# Autodesk Inventor assembly: BedAssembly
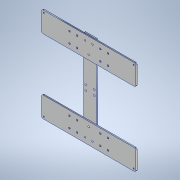
[picture p0: Inventor's stored thumbnail of the model, 180x180]
Saved by Autodesk Inventor 2020.2 (Build 242310000, 310)
## iProperties
Created: 2020-08-19
Part Number: BedAssembly
Document SubType Name: Assembly
Designer: JK
Author: JK
## Documents named in this file (3)
- C:\Users\JK\Documents\Inventor\Anet Upgrade\BedAssembly.iam
- C:\Users\JK\Documents\Inventor\Anet Upgrade\BedCarriageA.ipt
- C:\Users\JK\Documents\Inventor\Anet Upgrade\BedCarriageB.ipt
## Components (2 placed, 2 different names)
1. BedCarriageA:1 — Mate:1, Mate:2, Flush:1
2. BedCarriageB:1 — Mate:1, Mate:2, Flush:1
## Relationships (3: Mate 2, Flush 1)
- Mate:1: BedCarriageA:1 ↔ BedCarriageB:1
- Mate:2: BedCarriageA:1 ↔ BedCarriageB:1
- Flush:1: BedCarriageA:1 ↔ BedCarriageB:1
